# Autodesk Inventor assembly: 4in Plaction
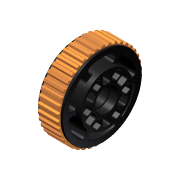
[picture p0: Inventor's stored thumbnail of the model, 180x180]
Saved by Autodesk Inventor 2011 (Build 150239000, 239)
## iProperties
Created: 2011-07-04
Part Number: 4in Plaction
Document SubType Name: Assembly
Designer: Dan Niemitalo
Author: Dan Niemitalo
## Documents named in this file (3)
- H:\Nemo\Documents\Robotics\COTS Parts\Wheels\4in Plaction.iam
- H:\Nemo\Documents\Robotics\Wheels and Sprockets\4MW_d01.ipt
- H:\Nemo\Documents\Robotics\COTS Parts\Wheels\Performance Wheel Parts\Roughtop Tread.ipt
## Components (3 placed, 2 different names)
1. 4MW_d01:1 — Insert:1, Mate:1, Insert:2
2. 4MW_d01:2 — Insert:1, Mate:1
3. Roughtop Tread:1 — Insert:2
## Relationships (3: Insert 2, Mate 1)
- Insert:1: 4MW_d01:1 ↔ 4MW_d01:2
- Mate:1: 4MW_d01:1 ↔ 4MW_d01:2
- Insert:2: 4MW_d01:1 ↔ Roughtop Tread:1
